# Autodesk Inventor assembly: Intake motor + pulley & 2 inch compliant wheel left
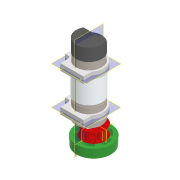
[picture p0: Inventor's stored thumbnail of the model, 180x180]
Saved by Autodesk Inventor 2020 (Build 240168000, 168)
## iProperties
Created: 2020-01-22
Part Number: Intake motor + pulley & 2 inch compliant wheel left
Document SubType Name: Assembly
Designer: ball
Author: ball
## Documents named in this file (3)
- C:\FTC\FTC8863CAD\2019 Robot\Collection\Intake\Intake motor + pulley & 2 inch compliant wheel left.iam
- C:\FTC\FTC8863CAD\2019 Robot\Collection\neverest 40 + mounts.iam
- C:\FTC\FTC8863CAD\2019 Robot\Collection\Intake\pulley 6mm bore + wheel.iam
## Components (2 placed, 2 different names)
1. neverest 40 + mounts:1 [sub-assembly] — Mate:1, Mate:2
2. pulley 6mm bore + wheel:1 [sub-assembly] — Mate:1, Mate:2
## Relationships (2: Mate 2)
- Mate:1: neverest 40 + mounts:1 ↔ pulley 6mm bore + wheel:1
- Mate:2: neverest 40 + mounts:1 ↔ pulley 6mm bore + wheel:1
